# Autodesk Inventor assembly: Montagem da base
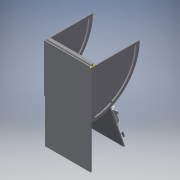
[picture p0: Inventor's stored thumbnail of the model, 180x180]
Saved by Autodesk Inventor 2019 (Build 230136000, 136)
## iProperties
Created: 2018-07-24
Part Number: Montagem da base
Material: Genérico
Document SubType Name: Assembly
Designer: Ernandes
Author: Ernandes
## Documents named in this file (5)
- C:\Users\Ernandes\Google Drive (sguimaraaes@gmail.com)\TCC\3D\lançador.inventor\base.inventor\Montagem da base.iam
- C:\Users\Ernandes\Google Drive (sguimaraaes@gmail.com)\TCC\3D\lançador.inventor\base.inventor\base base.ipt
- C:\Users\Ernandes\Google Drive (sguimaraaes@gmail.com)\TCC\3D\lançador.inventor\base.inventor\base.ipt
- C:\Users\Ernandes\Google Drive (sguimaraaes@gmail.com)\TCC\3D\lançador.inventor\base.inventor\arco base.ipt
- C:\Users\Ernandes\Google Drive (sguimaraaes@gmail.com)\TCC\3D\lançador.inventor\lançador.inventor\lançador.iam
## Components (5 placed, 4 different names)
1. base base:1 — Coincidência:1, Coincidência:2, Coincidência:3, Coincidência:4, Coincidência:5
2. base:1 — Coincidência:1
3. arco base:1 — Coincidência:2, Coincidência:3
4. arco base:2 — Coincidência:4, Coincidência:5
5. lançador:1 [sub-assembly]
## Relationships (5: Mate 5)
- Coincidência:1 [Mate] (-6 mm): base base:1 ↔ base:1
- Coincidência:2 [Mate] (5 mm): base base:1 ↔ arco base:1
- Coincidência:3 [Mate]: base base:1 ↔ arco base:1
- Coincidência:4 [Mate]: base base:1 ↔ arco base:2
- Coincidência:5 [Mate] (5 mm): base base:1 ↔ arco base:2
